# Autodesk Inventor assembly: WheelTyre624Bearing_MIR1
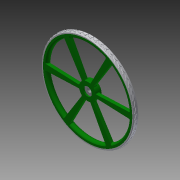
[picture p0: Inventor's stored thumbnail of the model, 180x180]
Saved by Autodesk Inventor 2014 SP1 (Build 180222100, 222)
## iProperties
Created: 2017-01-16
Part Number: WheelTyre624Bearing_MIR1
Document SubType Name: Assembly
Designer: danielsikar
Author: danielsikar
## Documents named in this file (4)
- C:\Users\danielsikar\Documents\Inventor\IoT-Trike\Assemblies\WheelTyre624Bearing_MIR1.iam
- C:\Users\danielsikar\Documents\Inventor\IoT-Trike\Parts\WheelDia120_MIR1.ipt
- C:\Users\danielsikar\Documents\Inventor\IoT-Trike\Parts\TyreR56mm_MIR1.ipt
- C:\Users\danielsikar\Documents\Inventor\IoT-Trike\Parts\624Bearing_MIR1.ipt
## Components (3 placed, 3 different names)
1. WheelDia120_MIR1:1 — Mate:2, Mate:1, Flush:1, Mate:3, Flush:2, Mate:4
2. TyreR56mm_MIR1:1 — Flush:1, Mate:3
3. 624Bearing_MIR1:1 — Flush:2, Mate:4
## Relationships (6: Flush 3, Mate 3)
- Mate:2 [Flush]: WheelDia120_MIR1:1
- Mate:1: WheelDia120_MIR1:1
- Flush:1: WheelDia120_MIR1:1 ↔ TyreR56mm_MIR1:1
- Mate:3: WheelDia120_MIR1:1 ↔ TyreR56mm_MIR1:1
- Flush:2: WheelDia120_MIR1:1 ↔ 624Bearing_MIR1:1
- Mate:4: WheelDia120_MIR1:1 ↔ 624Bearing_MIR1:1
